# Autodesk Inventor assembly: robot_base
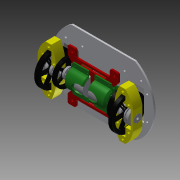
[picture p0: Inventor's stored thumbnail of the model, 180x180]
Saved by Autodesk Inventor 2014 SP1 (Build 180222100, 222)
## iProperties
Created: 2015-07-19
Part Number: robot_base
Document SubType Name: Assembly
Designer: astralien3000
Author: astralien3000
## Documents named in this file (4)
- C:\Users\astralien3000\Desktop\ceres\meca\v2016\robot_base.iam
- C:\Users\astralien3000\Desktop\ceres\meca\v2016\base.ipt
- C:\Users\astralien3000\Desktop\ceres\meca\v2016\odometer_block.iam
- C:\Users\astralien3000\Desktop\ceres\meca\v2016\wheel_block.iam
## Components (4 placed, 3 different names)
1. base:1 — Placage:1, Affleurement:1, Placage:3, Placage:4, Placage:5, Placage:6, Placage:7, Placage:8
2. odometer_block:1 [sub-assembly] — Placage:3, Placage:4
3. wheel_block:1 [sub-assembly] — Placage:5, Placage:6
4. wheel_block:2 [sub-assembly] — Placage:7, Placage:8
## Relationships (8: Mate 7, Flush 1)
- Placage:1 [Mate]: base:1
- Affleurement:1 [Flush]: base:1
- Placage:3 [Mate]: base:1 ↔ odometer_block:1
- Placage:4 [Mate]: base:1 ↔ odometer_block:1
- Placage:5 [Mate]: base:1 ↔ wheel_block:1
- Placage:6 [Mate]: base:1 ↔ wheel_block:1
- Placage:7 [Mate]: base:1 ↔ wheel_block:2
- Placage:8 [Mate]: base:1 ↔ wheel_block:2
